# Autodesk Inventor assembly: Base Design Robot 1
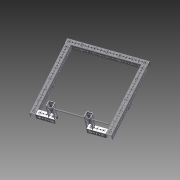
[picture p0: Inventor's stored thumbnail of the model, 180x180]
Saved by Autodesk Inventor 2015 (Build 190159000, 159)
## iProperties
Created: 2015-09-30
Part Number: Base Design Robot 1
Document SubType Name: Assembly
Designer: damedin
Author: damedin
## Documents named in this file (5)
- U:\Base Design Robot 1.iam
- U:\COTS Parts\Tetrix\Tetrix Channel 416mm.ipt
- U:\DropCenter Robot Part.ipt
- U:\COTS Parts\Tetrix\Tetrix channel 96mm.ipt
- U:\Rod.ipt
## Components (8 placed, 4 different names)
1. Tetrix Channel 416mm:2 — Mate:1, Flush:1, Mate:2, Mate:3, Flush:2, Mate:4
2. DropCenter Robot Part:1 — Mate:3, Flush:2, Mate:4, Mate:5, Flush:3, Mate:9
3. DropCenter Robot Part:2 — Mate:1, Flush:1, Mate:2, Mate:6, Mate:7, Flush:4, Mate:8
4. Tetrix channel 96mm:1 — Mate:5, Flush:3, Mate:9, Mate:10, Mate:11, Flush:7
5. Tetrix channel 96mm:2 — Mate:6, Mate:7, Flush:4, Mate:8, Mate:12, Flush:5, Flush:6
6. Tetrix channel 96mm:3 — Mate:10, Mate:11, Insert:1, Flush:7
7. Tetrix channel 96mm:4 — Mate:12, Flush:5, Flush:6
8. Rod:1 — Insert:1
## Relationships (20: Mate 12, Flush 7, Insert 1)
- Mate:1: Tetrix Channel 416mm:2 ↔ DropCenter Robot Part:2
- Flush:1: Tetrix Channel 416mm:2 ↔ DropCenter Robot Part:2
- Mate:2: Tetrix Channel 416mm:2 ↔ DropCenter Robot Part:2
- Mate:3: Tetrix Channel 416mm:2 ↔ DropCenter Robot Part:1
- Flush:2: Tetrix Channel 416mm:2 ↔ DropCenter Robot Part:1
- Mate:4: Tetrix Channel 416mm:2 ↔ DropCenter Robot Part:1
- Mate:5: DropCenter Robot Part:1 ↔ Tetrix channel 96mm:1
- Flush:3: DropCenter Robot Part:1 ↔ Tetrix channel 96mm:1
- Mate:6: DropCenter Robot Part:2 ↔ Tetrix channel 96mm:2
- Mate:7: DropCenter Robot Part:2 ↔ Tetrix channel 96mm:2
- Flush:4: DropCenter Robot Part:2 ↔ Tetrix channel 96mm:2
- Mate:8: DropCenter Robot Part:2 ↔ Tetrix channel 96mm:2
- Mate:9: DropCenter Robot Part:1 ↔ Tetrix channel 96mm:1
- Mate:10: Tetrix channel 96mm:1 ↔ Tetrix channel 96mm:3
- Mate:11: Tetrix channel 96mm:1 ↔ Tetrix channel 96mm:3
- Mate:12: Tetrix channel 96mm:2 ↔ Tetrix channel 96mm:4
- Flush:5: Tetrix channel 96mm:2 ↔ Tetrix channel 96mm:4
- Flush:6: Tetrix channel 96mm:2 ↔ Tetrix channel 96mm:4
- Insert:1: Tetrix channel 96mm:3 ↔ Rod:1
- Flush:7: Tetrix channel 96mm:1 ↔ Tetrix channel 96mm:3
